# Autodesk Inventor assembly: Assembly_Optical_Module
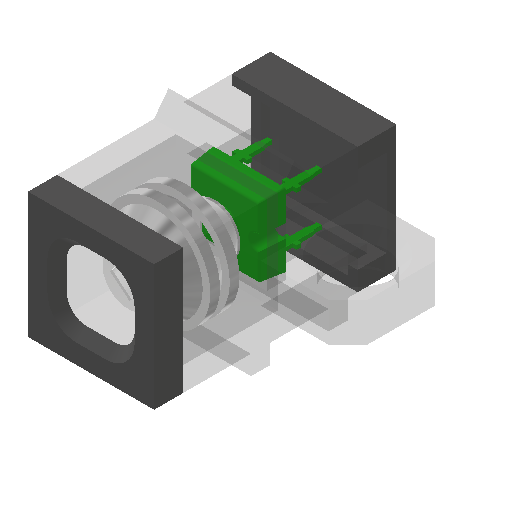
[picture p0: Inventor's stored thumbnail of the model, 512x512]
Saved by Autodesk Inventor 2026.1 (Build 301233020, 233B)
## iProperties
Created: 2026-01-26
Part Number: Assembly_Optical_Module
Document SubType Name: Assembly
Designer: samuel
Author: samuel
## Documents named in this file (6)
- E:\Fraunhofer\Design\Assembly_Optical_Module.iam
- E:\Fraunhofer\Design\Optical module_lid_2.ipt
- E:\Fraunhofer\Design\Optical module.ipt
- E:\Fraunhofer\Design\Optical module_lid.ipt
- E:\Fraunhofer\Design\Parts\LEN-R.ipt
- E:\Fraunhofer\Design\Parts\led-s-piranha-super-flux-rgb-for-kicad-1.snapshot.11\LED-PiranhaSuperFlux.3dshapes\Piranha Super Flux RGB LED 3mm\Piranha Super Flux RGB LED 3mm\Piranha Super Flux RGB LED 3mm.iam
## Components (6 placed, 5 different names)
1. Optical module_lid_2:1 — Flush:3, Flush:4, Mate:9
2. Optical module:1 — Mate:6, Mate:7, Mate:8, Flush:1, Flush:2, Flush:3, Flush:4, Mate:9, Mate:10
3. Optical module_lid:1 — Flush:1, Flush:2, Mate:10
4. LEN-R:1 — Mate:2, Mate:3, Mate:4, Mate:5
5. Piranha Super Flux RGB LED 3mm:1 [sub-assembly] — Mate:4, Mate:5, Mate:6, Mate:7, Mate:8
6. LEN-R:2 — Mate:2, Mate:3
## Relationships (13: Mate 9, Flush 4)
- Mate:2: LEN-R:1 ↔ LEN-R:2
- Mate:3 (1 mm): LEN-R:1 ↔ LEN-R:2
- Mate:4: LEN-R:1 ↔ Piranha Super Flux RGB LED 3mm:1
- Mate:5 (1 mm): LEN-R:1 ↔ Piranha Super Flux RGB LED 3mm:1
- Mate:6: Optical module:1 ↔ Piranha Super Flux RGB LED 3mm:1
- Mate:7: Optical module:1 ↔ Piranha Super Flux RGB LED 3mm:1
- Mate:8: Optical module:1 ↔ Piranha Super Flux RGB LED 3mm:1
- Flush:1: Optical module:1 ↔ Optical module_lid:1
- Flush:2: Optical module:1 ↔ Optical module_lid:1
- Flush:3: Optical module_lid_2:1 ↔ Optical module:1
- Flush:4: Optical module_lid_2:1 ↔ Optical module:1
- Mate:9: Optical module_lid_2:1 ↔ Optical module:1
- Mate:10: Optical module:1 ↔ Optical module_lid:1
